# Autodesk Inventor assembly: Right Rear Wheel with hub inside
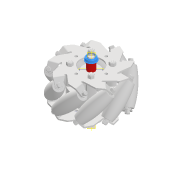
[picture p0: Inventor's stored thumbnail of the model, 180x180]
Saved by Autodesk Inventor 2020 (Build 240168000, 168)
## iProperties
Created: 2020-02-22
Part Number: Right Rear Wheel with hub inside
Document SubType Name: Assembly
Designer: ball
Author: ball
## Documents named in this file (11)
- C:\FTC\FTC8863CAD\2019 Robot\Mecanum Drive Train Metal\Right Rear Wheel with hub inside.iam
- C:\FTC\FTC8863CAD\GoBilda\1310 Parts\1310-0016-4008 assembly.ipt
- C:\FTC\FTC8863CAD\StepLibraries\Screws\M4 x 22 SOCKET HEAD CAP SCREW.ipt
- C:\FTC\FTC8863CAD\StepLibraries\Washers\M4 FLAT WASHER.ipt
- C:\FTC\FTC8863CAD\GoBilda\3213 Parts\3606-0000-0100 assembly.iam
- C:\FTC\FTC8863CAD\GoBilda\2102 Parts\2102-0008-0090.ipt
- C:\FTC\FTC8863CAD\GoBilda\3414 Parts\3414-4008-0016 assembly.iam
- C:\FTC\FTC8863CAD\GoBilda\1601 Parts\1601-0014-0008.ipt
- C:\FTC\FTC8863CAD\2019 Robot\Mecanum Drive Train Metal\spacer for inside of wheel.ipt
- C:\FTC\FTC8863CAD\2019 Robot\Mecanum Drive Train Metal\spacer for outside of wheel.ipt
- C:\FTC\FTC8863CAD\2019 Robot\Mecanum Drive Train Metal\spacer for wheel pulley.ipt
## Components (17 placed, 10 different names)
1. 3606-0000-0100 assembly:1 [sub-assembly] — Mate:26, Mate:27, Mate:28, Mate:29, Mate:30, Mate:31, Mate:40, Mate:41, Mate:42, Mate:43, Mate:45, Mate:46, Mate:54, Mate:56
2. M4 x 22 SOCKET HEAD CAP SCREW:6 — Mate:31
3. M4 FLAT WASHER:6 — Mate:30
4. 1310-0016-4008 assembly:2 — Mate:26, Mate:27, Mate:28, Mate:29, Mate:55, Mate:58
5. M4 x 22 SOCKET HEAD CAP SCREW:7 — Mate:43
6. M4 FLAT WASHER:7 — Mate:40
7. M4 x 22 SOCKET HEAD CAP SCREW:8 — Mate:46
8. M4 FLAT WASHER:8 — Mate:42
9. M4 x 22 SOCKET HEAD CAP SCREW:9 — Mate:45
10. M4 FLAT WASHER:9 — Mate:41
11. 2102-0008-0090:1 — Mate:54, Mate:55, Mate:59, Mate:61, Mate:63
12. 3414-4008-0016 assembly:1 [sub-assembly] — Mate:56, Flush:1, Mate:60, Mate:62
13. 1601-0014-0008:1 — Mate:64
14. 1601-0014-0008:2 — Flush:1, Mate:64
15. spacer for inside of wheel:1 — Mate:58, Mate:59
16. spacer for outside of wheel:1 — Mate:60, Mate:61
17. spacer for wheel pulley:1 — Mate:62, Mate:63
## Relationships (35: Mate 34, Flush 1)
- [Mate]: M4 x 22 SOCKET HEAD CAP SCREW:6 ↔ M4 FLAT WASHER:6
- [Mate]: M4 x 22 SOCKET HEAD CAP SCREW:6 ↔ M4 FLAT WASHER:6
- Mate:26: 3606-0000-0100 assembly:1 ↔ 1310-0016-4008 assembly:2
- Mate:27: 3606-0000-0100 assembly:1 ↔ 1310-0016-4008 assembly:2
- Mate:28: 3606-0000-0100 assembly:1 ↔ 1310-0016-4008 assembly:2
- Mate:29: 3606-0000-0100 assembly:1 ↔ 1310-0016-4008 assembly:2
- Mate:30: 3606-0000-0100 assembly:1 ↔ M4 FLAT WASHER:6
- Mate:31: 3606-0000-0100 assembly:1 ↔ M4 x 22 SOCKET HEAD CAP SCREW:6
- [Mate]: M4 x 22 SOCKET HEAD CAP SCREW:7 ↔ M4 FLAT WASHER:7
- [Mate]: M4 x 22 SOCKET HEAD CAP SCREW:7 ↔ M4 FLAT WASHER:7
- [Mate]: M4 x 22 SOCKET HEAD CAP SCREW:8 ↔ M4 FLAT WASHER:8
- [Mate]: M4 x 22 SOCKET HEAD CAP SCREW:8 ↔ M4 FLAT WASHER:8
- [Mate]: M4 x 22 SOCKET HEAD CAP SCREW:9 ↔ M4 FLAT WASHER:9
- [Mate]: M4 x 22 SOCKET HEAD CAP SCREW:9 ↔ M4 FLAT WASHER:9
- Mate:40: 3606-0000-0100 assembly:1 ↔ M4 FLAT WASHER:7
- Mate:41: 3606-0000-0100 assembly:1 ↔ M4 FLAT WASHER:9
- Mate:42: 3606-0000-0100 assembly:1 ↔ M4 FLAT WASHER:8
- Mate:43: 3606-0000-0100 assembly:1 ↔ M4 x 22 SOCKET HEAD CAP SCREW:7
- Mate:45: 3606-0000-0100 assembly:1 ↔ M4 x 22 SOCKET HEAD CAP SCREW:9
- Mate:46: 3606-0000-0100 assembly:1 ↔ M4 x 22 SOCKET HEAD CAP SCREW:8
- [Mate]: 2102-0008-0090:1 ↔ 3414-4008-0016 assembly:1
- [Mate]: 2102-0008-0090:1 ↔ 3414-4008-0016 assembly:1
- [Mate]: 2102-0008-0090:1 ↔ 1601-0014-0008:1
- [Mate]: 2102-0008-0090:1 ↔ 1601-0014-0008:2
- Mate:54: 3606-0000-0100 assembly:1 ↔ 2102-0008-0090:1
- Mate:55: 1310-0016-4008 assembly:2 ↔ 2102-0008-0090:1
- Mate:56 (1.27 mm): 3606-0000-0100 assembly:1 ↔ 3414-4008-0016 assembly:1
- Flush:1 (-3.0734 mm): 3414-4008-0016 assembly:1 ↔ 1601-0014-0008:2
- Mate:58: 1310-0016-4008 assembly:2 ↔ spacer for inside of wheel:1
- Mate:59: 2102-0008-0090:1 ↔ spacer for inside of wheel:1
- Mate:60: 3414-4008-0016 assembly:1 ↔ spacer for outside of wheel:1
- Mate:61: 2102-0008-0090:1 ↔ spacer for outside of wheel:1
- Mate:62: 3414-4008-0016 assembly:1 ↔ spacer for wheel pulley:1
- Mate:63: 2102-0008-0090:1 ↔ spacer for wheel pulley:1
- Mate:64 (-77.6732 mm): 1601-0014-0008:1 ↔ 1601-0014-0008:2
## Named parameters: d56_d39_d14_d12 = 0 mm, d57_d40_d15_d13 = 0 mm, d64_d56_d39_d14_d12 = 0 mm, d65_d57_d40_d15_d13 = 0 mm, d66_d56_d39_d14_d12 = 0 mm, d67_d57_d40_d15_d13 = 0 mm, d68_d56_d39_d14_d12 = 0 mm, d69_d57_d40_d15_d13 = 0 mm
